# Autodesk Inventor assembly: LeftTractionWheelsDTA
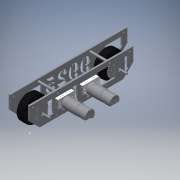
[picture p0: Inventor's stored thumbnail of the model, 180x180]
Saved by Autodesk Inventor 2017 (Build 210142000, 142)
## iProperties
Created: 2017-08-16
Part Number: LeftTractionWheelsDTA
Document SubType Name: Assembly
Designer: User
Author: User
## Documents named in this file (11)
- C:\Robotics\CAD\2016-17_CAD\Sub-Assemblies\LeftTractionWheelsDTA.iam
- C:\Robotics\CAD\2016-17_CAD\DriveTrain\drive train standoff.ipt
- C:\Robotics\CAD\2016-17_CAD\DriveTrain\DrainTrainPlate2.0LeftOutside.iam
- C:\Robotics\CAD\2016-17_CAD\DriveTrain\DriveTrainPlate2.0LeftInside.ipt
- C:\Robotics\CAD\COTSParts\Motors\Andymark 2964  NeveRest 40 Motor.ipt
- C:\Robotics\CAD\COTSParts\Tetrix\tetrix-motor-mounts-1.snapshot.1\Tetrex 2pc motor mount.ipt
- C:\Robotics\CAD\COTSParts\Actobotics\615 parts\615114.ipt
- C:\Robotics\CAD\COTSParts\Actobotics\545 parts\545456.ipt
- C:\Robotics\CAD\COTSParts\Actobotics\545 parts\545556.ipt
- C:\Robotics\CAD\COTSParts\Actobotics\634 parts\634080.ipt
- C:\Robotics\CAD\COTSParts\Wheels\4in Wheel Intergreated Hub 8mm Rev2.ipt
## Components (27 placed, 10 different names)
1. drive train standoff:1 — Mate:46, Mate:47
2. drive train standoff:2 — Mate:50, Mate:51
3. drive train standoff:3 — Mate:48, Mate:49
4. DrainTrainPlate2.0LeftOutside:1 [sub-assembly] — Mate:30, Flush:1, Mate:31, Flush:2, Flush:3, Mate:47, Mate:48, Mate:50
5. DriveTrainPlate2.0LeftInside:1 — Mate:28, Mate:29, Flush:1, Mate:32, Mate:33, Mate:44, Mate:45, Mate:46, Mate:49, Mate:51, Mate:56, Mate:57, Mate:58, Mate:59
6. Tetrex 2pc motor mount:1 — Mate:57, Mate:58, Mate:59, Mate:60, Flush:9
7. Tetrex 2pc motor mount:2 — Mate:44, Mate:45, Mate:52, Flush:6, Mate:56
8. 615114:1 — Mate:6, Mate:7, Mate:29, Flush:11
9. 615114:2 — Flush:10, Mate:62, Flush:11
10. 615114:3 — Mate:17, Mate:18, Mate:32, Flush:5, Flush:7
11. 615114:4 — Flush:5, Flush:7, Flush:8, Mate:54
12. 545456:1 — Mate:19, Mate:20, Mate:21
13. 545456:2 — Mate:13, Mate:14, Mate:15
14. 545456:3 — Mate:2, Mate:3, Mate:4
15. 545456:4 — Mate:8, Mate:9, Mate:25
16. 545556:1 — Mate:15, Mate:16, Mate:17
17. 545556:2 — Mate:4, Mate:5, Mate:6
18. 545556:3 — Flush:10, Mate:61, Mate:62
19. 545556:4 — Flush:8, Mate:53, Mate:54, Mate:55
20. 634080:1 — Mate:12, Mate:14, Mate:16, Mate:18, Mate:20, Mate:22, Mate:33, Flush:3
21. 634080:2 — Mate:1, Mate:3, Mate:5, Mate:7, Mate:9, Mate:26, Mate:28, Mate:31, Flush:2
22. 545556:6 — Mate:21, Mate:22
23. 4in Wheel Intergreated Hub 8mm Rev2:1 — Mate:1, Mate:2, Mate:8
24. 4in Wheel Intergreated Hub 8mm Rev2:2 — Mate:12, Mate:13, Mate:19
25. 545556:7 — Mate:25, Mate:26, Mate:30
26. Andymark 2964  NeveRest 40 Motor:3 — Mate:52, Flush:6, Mate:53, Mate:55
27. Andymark 2964  NeveRest 40 Motor:4 — Mate:60, Flush:9, Mate:61
## Relationships (57: Mate 47, Flush 10)
- Mate:1: 634080:2 ↔ 4in Wheel Intergreated Hub 8mm Rev2:1
- Mate:2: 545456:3 ↔ 4in Wheel Intergreated Hub 8mm Rev2:1
- Mate:3: 545456:3 ↔ 634080:2
- Mate:4: 545456:3 ↔ 545556:2
- Mate:5: 545556:2 ↔ 634080:2
- Mate:6: 615114:1 ↔ 545556:2
- Mate:7: 615114:1 ↔ 634080:2
- Mate:8: 545456:4 ↔ 4in Wheel Intergreated Hub 8mm Rev2:1
- Mate:9: 545456:4 ↔ 634080:2
- Mate:12: 634080:1 ↔ 4in Wheel Intergreated Hub 8mm Rev2:2
- Mate:13: 545456:2 ↔ 4in Wheel Intergreated Hub 8mm Rev2:2
- Mate:14: 545456:2 ↔ 634080:1
- Mate:15: 545456:2 ↔ 545556:1
- Mate:16: 545556:1 ↔ 634080:1
- Mate:17: 615114:3 ↔ 545556:1
- Mate:18: 615114:3 ↔ 634080:1
- Mate:19: 545456:1 ↔ 4in Wheel Intergreated Hub 8mm Rev2:2
- Mate:20: 545456:1 ↔ 634080:1
- Mate:21: 545456:1 ↔ 545556:6
- Mate:22: 634080:1 ↔ 545556:6
- Mate:25: 545456:4 ↔ 545556:7
- Mate:26: 634080:2 ↔ 545556:7
- Mate:28: DriveTrainPlate2.0LeftInside:1 ↔ 634080:2
- Mate:29 (6.35 mm): DriveTrainPlate2.0LeftInside:1 ↔ 615114:1
- Mate:30 (6.35 mm): DrainTrainPlate2.0LeftOutside:1 ↔ 545556:7
- Flush:1: DrainTrainPlate2.0LeftOutside:1 ↔ DriveTrainPlate2.0LeftInside:1
- Mate:31: DrainTrainPlate2.0LeftOutside:1 ↔ 634080:2
- Flush:2: DrainTrainPlate2.0LeftOutside:1 ↔ 634080:2
- Mate:32 (6.35 mm): DriveTrainPlate2.0LeftInside:1 ↔ 615114:3
- Mate:33: DriveTrainPlate2.0LeftInside:1 ↔ 634080:1
- Flush:3: DrainTrainPlate2.0LeftOutside:1 ↔ 634080:1
- Mate:44: DriveTrainPlate2.0LeftInside:1 ↔ Tetrex 2pc motor mount:2
- Mate:45: DriveTrainPlate2.0LeftInside:1 ↔ Tetrex 2pc motor mount:2
- Flush:5: 615114:3 ↔ 615114:4
- Mate:46: drive train standoff:1 ↔ DriveTrainPlate2.0LeftInside:1
- Mate:47: drive train standoff:1 ↔ DrainTrainPlate2.0LeftOutside:1
- Mate:48: drive train standoff:3 ↔ DrainTrainPlate2.0LeftOutside:1
- Mate:49: drive train standoff:3 ↔ DriveTrainPlate2.0LeftInside:1
- Mate:50: drive train standoff:2 ↔ DrainTrainPlate2.0LeftOutside:1
- Mate:51: drive train standoff:2 ↔ DriveTrainPlate2.0LeftInside:1
- Mate:52: Tetrex 2pc motor mount:2 ↔ Andymark 2964  NeveRest 40 Motor:3
- Flush:6: Tetrex 2pc motor mount:2 ↔ Andymark 2964  NeveRest 40 Motor:3
- Flush:7: 615114:3 ↔ 615114:4
- Flush:8: 615114:4 ↔ 545556:4
- Mate:53: 545556:4 ↔ Andymark 2964  NeveRest 40 Motor:3
- Mate:54: 615114:4 ↔ 545556:4
- Mate:55: 545556:4 ↔ Andymark 2964  NeveRest 40 Motor:3
- Mate:56: DriveTrainPlate2.0LeftInside:1 ↔ Tetrex 2pc motor mount:2
- Mate:57: DriveTrainPlate2.0LeftInside:1 ↔ Tetrex 2pc motor mount:1
- Mate:58: DriveTrainPlate2.0LeftInside:1 ↔ Tetrex 2pc motor mount:1
- Mate:59: DriveTrainPlate2.0LeftInside:1 ↔ Tetrex 2pc motor mount:1
- Mate:60: Tetrex 2pc motor mount:1 ↔ Andymark 2964  NeveRest 40 Motor:4
- Flush:9: Tetrex 2pc motor mount:1 ↔ Andymark 2964  NeveRest 40 Motor:4
- Flush:10: 615114:2 ↔ 545556:3
- Mate:61: 545556:3 ↔ Andymark 2964  NeveRest 40 Motor:4
- Mate:62: 615114:2 ↔ 545556:3
- Flush:11: 615114:1 ↔ 615114:2
